# Autodesk Inventor assembly: Shaft Collar Metal
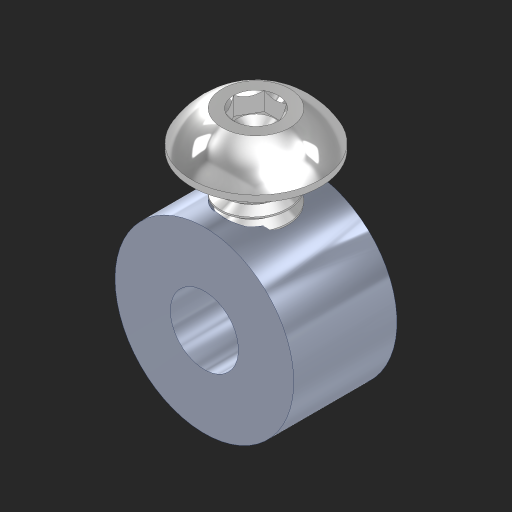
[picture p0: Inventor's stored thumbnail of the model, 512x512]
Saved by Autodesk Inventor 2023 (Build 270158000, 158)
## iProperties
Created: 2022-08-01
Part Number: Shaft Collar Metal
Document SubType Name: Assembly
Designer: ylu12
Author: ylu12
## Documents named in this file (5)
- C:\Users\ylu12\Documents\GitHub\VEX-CAD-Inventor\Motion\Shaft Collar Metal\Shaft Collar Hex Threaded.iam
- C:\Users\ylu12\Documents\GitHub\VEX-CAD-Inventor\Motion\Shaft Collar without Set Screw.ipt
- C:\Users\ylu12\Documents\GitHub\VEX-CAD-Inventor\Structure\Hardware\Screw Steel - Hex\SScrew Hex Threaded .250.ipt
- C:\Users\ylu12\Documents\GitHub\VEX-CAD-Inventor\Structure\Hardware\Screw Steel - Hex.ipt
- C:\Users\ylu12\Documents\GitHub\VEX-CAD-Inventor\Motion\Shaft Collar Metal.iam
## Components (2 placed, 2 different names)
1. Shaft Collar without Set Screw:1 — Mate:1, Mate:2, Flush:1, Insert:2
2. SScrew Hex Threaded .250:1 — Insert:2
## Relationships (4: Mate 2, Flush 1, Insert 1)
- Mate:1: Shaft Collar without Set Screw:1
- Mate:2: Shaft Collar without Set Screw:1
- Flush:1: Shaft Collar without Set Screw:1
- Insert:2 (2.54 mm): Shaft Collar without Set Screw:1 ↔ SScrew Hex Threaded .250:1
